# Autodesk Inventor assembly: ASY PNS 1730 elbow
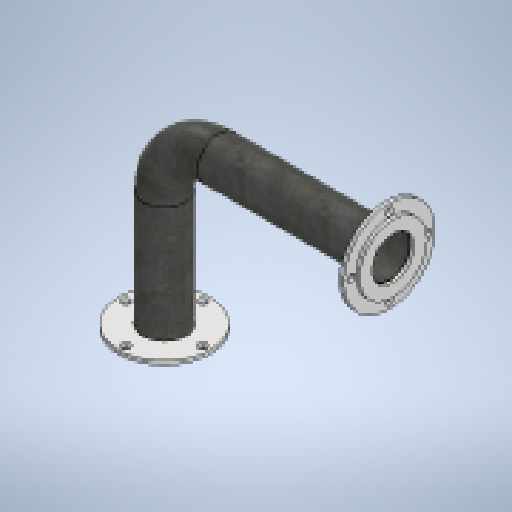
[picture p0: Inventor's stored thumbnail of the model, 512x512]
Saved by Autodesk Inventor 2025.1 (Build 291241020, 241B)
## iProperties
Created: 2025-07-04
Part Number: ASY PNS 1730 elbow
Document SubType Name: Assembly
Designer: user
Author: user
## Documents named in this file (6)
- C:\Users\user\YandexDisk-badmisterfox\home pc\Inventor\PNS2-Panaevsk\Filter D1200\ASY PNS 1730 elbow.iam
- C:\Users\user\YandexDisk-badmisterfox\home pc\Inventor\PNS2-Panaevsk\CC\en-US\JIS B 2312 90 (2)\JIS B 2312 90 Deg Long Elbow Steel 80A x Sch 40.ipt
- C:\Users\user\YandexDisk-badmisterfox\home pc\Inventor\PNS2-Panaevsk\Filter D1200\PNS 1733 FDS tube 3.ipt
- C:\Users\user\YandexDisk-badmisterfox\home pc\Inventor\PNS2-Panaevsk\Filter D1200\PNS 1721 FDS flange DN90.ipt
- C:\Users\user\YandexDisk-badmisterfox\home pc\Inventor\PNS2-Panaevsk\Filter D1200\PNS 1732 FDS free flange DN90.ipt
- C:\Users\user\YandexDisk-badmisterfox\home pc\Inventor\PNS2-Panaevsk\Filter D1200\PNS 756 FDS tube.ipt
## Components (7 placed, 5 different names)
1. JIS B 2312 90 Deg Long Elbow Steel 80A x Sch 40.ipt:1
2. PNS 1733 FDS tube 3.ipt:1
3. PNS 1721 FDS flange DN90.ipt:1
4. PNS 1732 FDS free flange DN90.ipt:1
5. PNS 756 FDS tube.ipt:1
6. PNS 1721 FDS flange DN90.ipt:2
7. PNS 1732 FDS free flange DN90.ipt:2
## Relationships (6: WeldJoint 6)
- [WeldJoint]: PNS 1733 FDS tube 3.ipt:1 ↔ PNS 1732 FDS free flange DN90.ipt:1
- [WeldJoint]: PNS 1733 FDS tube 3.ipt:1 ↔ PNS 1721 FDS flange DN90.ipt:1
- [WeldJoint]: JIS B 2312 90 Deg Long Elbow Steel 80A x Sch 40.ipt:1 ↔ PNS 1733 FDS tube 3.ipt:1
- [WeldJoint]: JIS B 2312 90 Deg Long Elbow Steel 80A x Sch 40.ipt:1 ↔ PNS 756 FDS tube.ipt:1
- [WeldJoint]: PNS 756 FDS tube.ipt:1 ↔ PNS 1732 FDS free flange DN90.ipt:2
- [WeldJoint]: PNS 1721 FDS flange DN90.ipt:2 ↔ PNS 1732 FDS free flange DN90.ipt:2
